# Autodesk Inventor assembly: B30041_ASSY
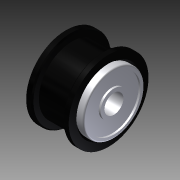
[picture p0: Inventor's stored thumbnail of the model, 180x180]
Saved by Autodesk Inventor 2013 SP2 (Build 170200200, 200)
## iProperties
Created: 2012-01-24
Part Number: B30041_ASSY
Document SubType Name: Assembly
Designer: ERF
Catalog Web Link: varies
Description: Smooth Idler Assembly
Vendor: custom
Stock Number: B30041_ASM
Mass: 2.21849 g
Surface Area: 41.2914 cm^2
Volume: 1.85724 cm^3
Density: 1.19451 g/cm^3
Author: ERF
## Documents named in this file (4)
- C:\Users\Edward\Desktop\Shapeoko_v2\B30041.iam
- C:\Users\Edward\Desktop\Shapeoko_v2\BEARING_5_16_5.ipt
- C:\Users\Edward\Desktop\Shapeoko_v2\B18026.ipt
- C:\Users\Edward\Desktop\Shapeoko_v2\B17023.ipt
## Components (4 placed, 3 different names)
1. B18026:2 — Insert:2, Insert:3
2. BEARING_5_16_5:3 — Insert:3
3. BEARING_5_16_5:4 — Insert:1, Insert:2
4. B17023:2 — Insert:1
## Relationships (3: Insert 3)
- Insert:1: BEARING_5_16_5:4 ↔ B17023:2
- Insert:2: B18026:2 ↔ BEARING_5_16_5:4
- Insert:3: B18026:2 ↔ BEARING_5_16_5:3
